# Autodesk Inventor assembly: AN929-3D
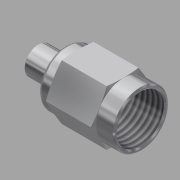
[picture p0: Inventor's stored thumbnail of the model, 180x180]
Saved by Autodesk Inventor 2019 (Build 230136000, 136)
## iProperties
Created: 2018-11-23
Part Number: AN929-3D
Document SubType Name: Assembly
Designer: erics
Mass: 2.76149 g
Surface Area: 15.2423 cm^2
Volume: 0.990042 cm^3
Density: 2.78927 g/cm^3
Author: erics
## Documents named in this file (6)
- D:\Users\erics\Documents\CAD Library\Pipe Fittings\AN-MS-Fittings\AN929\AN929-3D.iam
- D:\Users\erics\Documents\CAD Library\Pipe Fittings\AN-MS-Fittings\AN929.ipt
- D:\Users\erics\Documents\CAD Library\Pipe Fittings\AN-MS-Fittings\AN818.ipt
- D:\Users\erics\Documents\CAD Library\Pipe Fittings\AN-MS-Fittings\AN929.iam
- D:\Users\erics\Documents\CAD Library\Pipe Fittings\AN-MS-Fittings\AN929\AN929-3D.ipt
- D:\Users\erics\Documents\CAD Library\Pipe Fittings\AN-MS-Fittings\AN818\AN818-3D.ipt
## Components (2 placed, 2 different names)
1. AN929-3D:1 — Insert:1
2. AN818-3D:1 — Insert:1
## Relationships (1: Insert 1)
- Insert:1: AN929-3D:1 ↔ AN818-3D:1
